# Autodesk Inventor assembly: arm
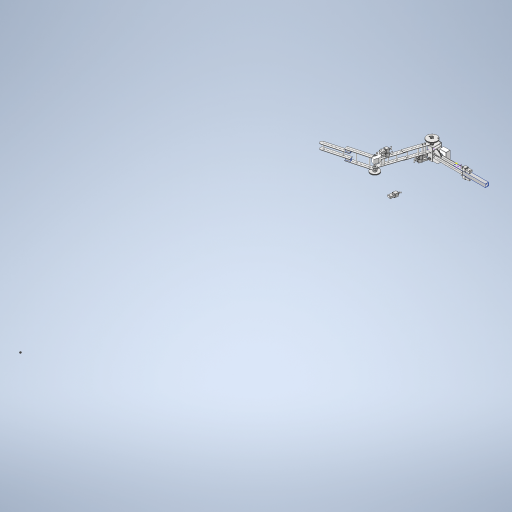
[picture p0: Inventor's stored thumbnail of the model, 512x512]
Saved by Autodesk Inventor 2024 (Build 280153000, 153)
## iProperties
Created: 2025-08-05
Part Number: arm
Document SubType Name: Assembly
Designer: HosodaLab2
Author: HosodaLab2
## iProperties of the stored document CSH-SUS-M6-130.ipt
Created: 2014-02-13
Part Number: CSH-SUS-M6-130
Material: 一般
Document SubType Name: Modeling
Designer: HosodaLab2
Density: 1 g/cm^3
Appearance: 既定
Sending System: SolidWorks 2007
Last Author: guan-li
Last Saved: 2014-03-10
Author: HosodaLab2
## Documents named in this file (68)
- C:\Users\HosodaLab2\OneDrive - Kyoto University\ドキュメント\Inventor\arm2\arm.iam
- C:\Users\HosodaLab2\OneDrive - Kyoto University\ドキュメント\Inventor\arm2\arm_jig.ipt
- C:\Users\HosodaLab2\OneDrive - Kyoto University\ドキュメント\Inventor\arm2\elbow_stopper.ipt
- C:\Users\HosodaLab2\OneDrive - Kyoto University\ドキュメント\Inventor\arm2\base.ipt
- C:\Users\HosodaLab2\OneDrive - Kyoto University\ドキュメント\Inventor\arm2\elbow_lower_plate.ipt
- C:\Users\HosodaLab2\OneDrive - Kyoto University\ドキュメント\Inventor\arm2\elbow_upper_plate.ipt
- C:\Users\HosodaLab2\OneDrive - Kyoto University\ドキュメント\Inventor\arm2\shoulder_stopper.ipt
- C:\Users\HosodaLab2\OneDrive - Kyoto University\ドキュメント\Inventor\arm2\CUI_AMT102-1024-I8000-S.iam
- C:\Users\HosodaLab2\OneDrive - Kyoto University\ドキュメント\Inventor\arm2\STHRANG8-MB.iam
- C:\Users\HosodaLab2\OneDrive - Kyoto University\ドキュメント\Inventor\arm2\F686ZZ.ipt
- C:\Users\HosodaLab2\OneDrive - Kyoto University\ドキュメント\Inventor\arm2\shoulder1_shaft.ipt
- C:\Users\HosodaLab2\OneDrive - Kyoto University\ドキュメント\Inventor\arm2\elbow_shaft.ipt
- C:\Users\HosodaLab2\OneDrive - Kyoto University\ドキュメント\Inventor\arm2\pully_elbow.ipt
- C:\Users\HosodaLab2\OneDrive - Kyoto University\ドキュメント\Inventor\arm2\pully_shoulder1.ipt
- C:\Users\HosodaLab2\OneDrive - Kyoto University\ドキュメント\Inventor\arm2\shoulder1_upper_plate.ipt
- C:\Users\HosodaLab2\OneDrive - Kyoto University\ドキュメント\Inventor\arm2\shoulder1_shaftholder_spacer_bottom.ipt
- C:\Users\HosodaLab2\OneDrive - Kyoto University\ドキュメント\Inventor\arm2\shoulder1_shaftholder_spacer_upper.ipt
- C:\Users\HosodaLab2\OneDrive - Kyoto University\ドキュメント\Inventor\arm2\shoulder1_upper_enocder_spacer.ipt
- C:\Users\HosodaLab2\OneDrive - Kyoto University\ドキュメント\Inventor\arm2\shoulder1_under_lower_plate_spacer.ipt
- C:\Users\HosodaLab2\OneDrive - Kyoto University\ドキュメント\Inventor\arm2\shoulder1_lower_cover.ipt
- C:\Users\HosodaLab2\OneDrive - Kyoto University\ドキュメント\Inventor\arm2\shoulder1_upper_cover.ipt
- C:\Users\HosodaLab2\OneDrive - Kyoto University\ドキュメント\Inventor\arm2\STHRANG10-MB_ss.ipt
- C:\Users\HosodaLab2\OneDrive - Kyoto University\ドキュメント\Inventor\arm2\shoulder1_lower_plate.ipt
- C:\Users\HosodaLab2\OneDrive - Kyoto University\ドキュメント\Inventor\arm2\F688ZZ.iam
- C:\Users\HosodaLab2\OneDrive - Kyoto University\ドキュメント\Inventor\arm2\SCST6-8.iam
- C:\Users\HosodaLab2\OneDrive - Kyoto University\ドキュメント\Inventor\arm2\shoulder2_upper_plate_spacer.ipt
- C:\Users\HosodaLab2\OneDrive - Kyoto University\ドキュメント\Inventor\arm2\shoulder1_encorder_spacer.ipt
- C:\Users\HosodaLab2\OneDrive - Kyoto University\ドキュメント\Inventor\arm2\shoulder2_pully_spacer.ipt
- C:\Users\HosodaLab2\OneDrive - Kyoto University\ドキュメント\Inventor\arm2\pully_shoulder2.ipt
- pully_shoulder_2_80.ipt
- C:\Users\HosodaLab2\OneDrive - Kyoto University\ドキュメント\Inventor\arm2\shoulder2_upperplate_left_spacer.ipt
- C:\Users\HosodaLab2\OneDrive - Kyoto University\ドキュメント\Inventor\arm2\shoulder2_upperplate_right_spacer.ipt
- C:\Users\HosodaLab2\OneDrive - Kyoto University\ドキュメント\Inventor\arm2\shoulder2_lower_left_plate.ipt
- C:\Users\HosodaLab2\OneDrive - Kyoto University\ドキュメント\Inventor\arm2\shoulder2_lower_right_plate.ipt
- C:\Users\HosodaLab2\OneDrive - Kyoto University\ドキュメント\Inventor\arm2\elbow_encorder_spacer.ipt
- C:\Users\HosodaLab2\OneDrive - Kyoto University\ドキュメント\Inventor\arm2\elbow_upperplate_left_spacer.ipt
- C:\Users\HosodaLab2\OneDrive - Kyoto University\ドキュメント\Inventor\arm2\elbow_upperplate_right_spacer.ipt
- C:\Users\HosodaLab2\OneDrive - Kyoto University\ドキュメント\Inventor\arm2\elbow_pully_spacer.ipt
- C:\Users\HosodaLab2\OneDrive - Kyoto University\ドキュメント\Inventor\arm2\shoulder2_lower_plate_spacer.ipt
- C:\Users\HosodaLab2\OneDrive - Kyoto University\ドキュメント\Inventor\arm2\elbow_lower_plate_spacer.ipt
- C:\Users\HosodaLab2\OneDrive - Kyoto University\ドキュメント\Inventor\arm2\elbow_upper_plate_spacer.ipt
- C:\Users\HosodaLab2\OneDrive - Kyoto University\ドキュメント\Inventor\arm2\shoulder1_NewPart2.ipt
- **C:\Users\HosodaLab2\OneDrive - Kyoto University\ドキュメント\Inventor\arm2\arm.iam*LocalDocs*xAaaaalcaAaaaaaaaAaaaqn4oUb*CSH-SUS-M6-130.ipt
- C:\Users\HosodaLab2\OneDrive - Kyoto University\ドキュメント\Inventor\arm2\shoulder2_elbow_strain_sensor_near.iam
- C:\Users\HosodaLab2\OneDrive - Kyoto University\ドキュメント\Inventor\arm2\shoulder2_elbow_strain_sensor_away.iam
- C:\Users\HosodaLab2\OneDrive - Kyoto University\ドキュメント\Inventor\arm2\shoulder2_shaft.ipt
- C:\Users\HosodaLab2\OneDrive - Kyoto University\ドキュメント\Inventor\arm2\shoulder2_lower_plate_bolt_spcaer.ipt
- C:\Users\HosodaLab2\OneDrive - Kyoto University\ドキュメント\Inventor\arm2\shoulder2_uppper_plate_bolt_spcaer.ipt
- C:\Users\HosodaLab2\OneDrive - Kyoto University\ドキュメント\Inventor\arm2\strain_sensor_spacer.ipt
- C:\Users\HosodaLab2\OneDrive - Kyoto University\ドキュメント\Inventor\arm2\shoulder1_strain_sensor.iam
- C:\Users\HosodaLab2\OneDrive - Kyoto University\ドキュメント\Inventor\arm2\shoulder1_strain_sensor_spacer.ipt
- C:\Users\HosodaLab2\OneDrive - Kyoto University\ドキュメント\Inventor\arm2\shoulder2_shaftholder_spacer_upper.ipt
- C:\Users\HosodaLab2\OneDrive - Kyoto University\ドキュメント\Inventor\arm2\3dprint\pully_elbow_40.ipt
- C:\Users\HosodaLab2\OneDrive - Kyoto University\ドキュメント\Inventor\arm2\3dprint\pully_elbow_50.ipt
- C:\Users\HosodaLab2\OneDrive - Kyoto University\ドキュメント\Inventor\arm2\SCST8-8.iam
- C:\Users\HosodaLab2\OneDrive - Kyoto University\ドキュメント\Inventor\arm2\shoulder2_upper_plate_left.ipt
- C:\Users\HosodaLab2\OneDrive - Kyoto University\ドキュメント\Inventor\arm2\shoulder2_upper_plate_rigth.ipt
- shoulder2_upper_plate_rigtht.ipt
- C:\Users\HosodaLab2\OneDrive - Kyoto University\ドキュメント\Inventor\arm2\shoulder2_encorder_spacer.ipt
- C:\Users\HosodaLab2\OneDrive - Kyoto University\ドキュメント\Inventor\arm2\shoulder2_shaftholder_spacer.ipt
- C:\Users\HosodaLab2\OneDrive - Kyoto University\ドキュメント\Inventor\arm2\shoulder1_verticval_cover.ipt
- C:\Users\HosodaLab2\OneDrive - Kyoto University\ドキュメント\Inventor\arm2\pully_shoulder2_70.ipt
- C:\Users\HosodaLab2\OneDrive - Kyoto University\ドキュメント\Inventor\arm2\pully_shoulder2_90ipt.ipt
- C:\Users\HosodaLab2\OneDrive - Kyoto University\ドキュメント\Inventor\arm2\pully_shoulder2_100.ipt
- C:\Users\HosodaLab2\OneDrive - Kyoto University\ドキュメント\Inventor\Content Center Files\R2024\ja-JP\ISO 4762(2)\ISO 4762 - M3 x 16ISO.ipt
- C:\Users\HosodaLab2\OneDrive - Kyoto University\ドキュメント\Inventor\arm2\new_shoulder2_elbow_strain_sensor_away.iam
- **C:\Users\HosodaLab2\OneDrive - Kyoto University\ドキュメント\Inventor\arm\arm.iam*LocalDocs*xAaaaalcaAaaaaaaaAaaaqn4oUb*CSH-SUS-M6-130.ipt
- C:\Users\HosodaLab2\OneDrive - Kyoto University\ドキュメント\Inventor\arm2\CSH-SUS-M6-130.SLDPRT
## Components (102 placed, 60 different names)
1. arm_jig:1 — 回転:140, 回転:141, 回転:142, 回転:143
2. base:1 — 回転:34, 回転:74, 回転:217, 回転:218, 円柱状:21, 円柱状:22, メイト:10, 円柱状:23, 円柱状:24, メイト:11, 回転:225, 回転:226, 回転:227, 回転:228
3. elbow_lower_plate:1 — 回転:142, 回転:143, リジッド:2, 回転:167
4. elbow_stopper:1 — 回転:168, 回転:169
5. shoulder1_encorder_spacer:1 — 回転:62, 回転:63
6. shoulder_stopper:1 — 回転:58, 回転:59
7. shoulder1_plate:1 — 回転:34, 角度:3, 回転:58, 回転:59, 回転:62, 回転:63, 回転:89, 角度:5, 回転:217
8. elbow_upper_plate:2 — 回転:140, 回転:141, 回転:144, 回転:153, 回転:215, 回転:216
9. shoulder2_lower_left_plate:1 — 回転:132, 回転:133, 角度:9, 回転:152, 回転:182, 回転:183, 回転:184, 回転:185, 回転:219
10. shoulder2_upper_plate_left:1 — 回転:173, 回転:175, メイト:3, 回転:184, 回転:185, 回転:220, 回転:263
11. shoulder2_lower_right_plate:1 — 回転:106, 回転:151, 回転:168, 回転:169, メイト:5, 回転:186, 回転:187, 回転:190
12. shoulder2_upper_plate_rigtht:1 — 回転:186, 回転:187, 回転:200, 回転:201, 回転:202, 回転:203, 回転:245, 回転:262, 回転:266, 回転:267, 角度:10
13. arm_jig:2
14. elbow_lower_plate:3 — 回転:155, 回転:156
15. elbow_upper_plate:3 — 回転:154, 回転:161, 回転:162, 回転:163, 回転:166, リジッド:1
16. CUI_AMT102-1024-I8000-S:3 [sub-assembly] — 角度:3, 回転:87, 回転:92
17. F686ZZ:1
18. pully_elbow:1 — 回転:164, 回転:165
19. pully_shoulder1:3 — 回転:157, 回転:158
20. shoulder1_shaftholder_spacer_bottom:1 — 回転:79, 回転:121
21. shoulder1_shaftholder_spacer_upper:1 — 回転:83
22. shoulder1_upper_enocder_spacer:1 — 回転:87, 回転:95
23. shoulder1_under_lower_plate_spacer:1 — 回転:93, 回転:109
24. shoulder1_upper_cover:1 — 角度:5, 回転:95, 回転:231, 回転:235, 回転:236, 回転:274, 回転:275
25. shoulder1_verticval_cover:1 — 回転:235, 回転:236, 回転:237, 回転:238, 回転:259, 回転:282, メイト:16, メイト:18, メイト:20, 回転:283
26. STHRANG10-MB_ss:1 — 回転:79, 回転:83, 回転:157, 回転:158, メイト:9
27. STHRANG8-MB:2 [sub-assembly] — 円柱状:8, 回転:159, 回転:253, 回転:281, メイト:15
28. shoulder1_lower_plate:1 — 回転:74, 回転:88, 角度:7, 回転:218
29. F688ZZ:1 [sub-assembly] — 回転:88, 回転:93, 回転:121, 回転:211
30. shoulder2_upper_plate_spacer:1 — 回転:173, 回転:200
31. F688ZZ:3 [sub-assembly] — 回転:106, 回転:137
32. F688ZZ:4 [sub-assembly] — 回転:134, 回転:212
33. shoulder1_lower_cover:2 — 角度:7, 回転:109, 回転:237, 回転:238, 回転:242, 回転:243, 回転:244
34. pully_shoulder_2_80:1 — 円柱状:8, 回転:159
35. CUI_AMT102-1024-I8000-S:4 [sub-assembly] — 回転:134, 角度:9, 回転:136
36. elbow_encorder_spacer:1 — 回転:132, 回転:133
37. elbow_upperplate_right_spacer:1 — 回転:137, 回転:144
38. elbow_upperplate_left_spacer:2 — 回転:136, 回転:162
39. elbow_pully_spacer:1 — 回転:146, 回転:147, 回転:161, 回転:163
40. STHRANG8-MB:4 [sub-assembly] — 回転:146, 回転:147, 回転:164, 回転:165, メイト:7
41. STHRANG8-MB:5 [sub-assembly] — 回転:215, 回転:216
42. shoulder2_upper_plate_spacer:2 — 回転:175
43. shoulder2_lower_plate_spacer:1 — 回転:151
44. shoulder2_lower_plate_spacer:2 — 回転:152
45. elbow_lower_plate_spacer:1 — 回転:155, リジッド:2
46. elbow_upper_plate_spacer:1 — 回転:153, 回転:166
47. elbow_upper_plate_spacer:2 — 回転:154, リジッド:1
48. elbow_lower_plate_spacer:2 — 回転:156, 回転:167
49. shoulder1_NewPart2:1
50. shoulder2_elbow_strain_sensor_near:1 [sub-assembly] — メイト:3, メイト:4, 円柱状:17, 円柱状:18, 回転:222
51. CSH-SUS-M6-130:1 — 回転:202, 円柱状:18, 円柱状:20
52. CSH-SUS-M6-130:2 — 回転:201, 円柱状:17, 円柱状:19
53. CSH-SUS-M6-130:3 — 回転:183, 円柱状:14, 円柱状:16
54. CSH-SUS-M6-130:4 — 回転:182, 円柱状:13, 円柱状:15
55. shoulder2_elbow_strain_sensor_away:1 [sub-assembly] — メイト:4, 円柱状:19, 円柱状:20, 回転:221
56. shoulder2_elbow_strain_sensor_away:2 [sub-assembly] — 円柱状:15, 円柱状:16, メイト:6
57. shoulder2_elbow_strain_sensor_near:2 [sub-assembly] — 円柱状:13, 円柱状:14, メイト:5, メイト:6, 回転:223, 回転:224
58. shoulder2_uppper_plate_bolt_spcaer:1 — 回転:203
59. shoulder2_lower_plate_bolt_spcaer:1 — 回転:190
60. shoulder1_shaft:1 — 回転:211, メイト:9, 円柱状:25, 回転:241
61. elbow_shaft:1 — 回転:212, メイト:7
62. shoulder2_shaft:1 — 回転:282, 円柱状:26, 円柱状:27, メイト:15
63. shoulder2_lower_plate_bolt_spcaer:2 — 回転:219
64. shoulder2_uppper_plate_bolt_spcaer:2 — 回転:220
65. strain_sensor_spacer:1 — 回転:221
66. strain_sensor_spacer:2 — 回転:222
67. strain_sensor_spacer:3 — 回転:223
68. strain_sensor_spacer:4 — 回転:224
69. shoulder1_strain_sensor:1 [sub-assembly] — 円柱状:21, 円柱状:22, メイト:10
70. shoulder1_strain_sensor:2 [sub-assembly] — 円柱状:23, 円柱状:24, メイト:11
71. shoulder1_strain_sensor_spacer:1 — 回転:225
72. shoulder1_strain_sensor_spacer:2 — 回転:228
73. shoulder1_strain_sensor_spacer:3 — 回転:226
74. shoulder1_strain_sensor_spacer:4 — 回転:227
75. F688ZZ:2 [sub-assembly] — 回転:89, 回転:92
76. STHRANG8-MB:6 [sub-assembly] — 円柱状:25, 回転:231
77. shoulder2_shaftholder_spacer_upper:1
78. STHRANG8-MB:9 [sub-assembly] — 回転:241, 回転:242
79. SCST6-8:1 [sub-assembly] — 回転:243, 回転:244
80. pully_elbow_40:1
81. pully_elbow_50:1
82. SCST8-8:1 [sub-assembly] — 回転:259, メイト:12, メイト:13, メイト:17, メイト:19, メイト:21, 回転:283
83. CUI_AMT102-1024-I8000-S:5 [sub-assembly] — 回転:245, 回転:246, 回転:268, 角度:10
84. F688ZZ:7 [sub-assembly] — 回転:262, 回転:265, 回転:268
85. shoulder2_pully_spacer:2 — 回転:246, 回転:253
86. shoulder2_upperplate_left_spacer:2 — 回転:279, 円柱状:27
87. shoulder2_upperplate_right_spacer:2 — 回転:265, メイト:12, 円柱状:26, メイト:13
88. SCST8-8:2 [sub-assembly] — 回転:276, 回転:278
89. F688ZZ:9 [sub-assembly] — 回転:263, 回転:264, 回転:271, 回転:273, 回転:279
90. STHRANG8-MB:10 [sub-assembly] — 回転:264
91. shoulder2_encorder_spacer:1 — 回転:266, 回転:267
92. shoulder2_shaftholder_spacer:1 — 回転:271
93. SCST8-8:3 [sub-assembly] — 回転:273
94. shoulder1_verticval_cover:2 — 回転:274, 回転:275, 回転:276, 回転:278
95. SCST8-8:4 [sub-assembly] — 回転:281
96. pully_shoulder_2_80:6
97. pully_shoulder_2_80:5
98. pully_shoulder_2_80:7
99. ISO 4762 M3 x 16:1 — メイト:16, メイト:17
100. ISO 4762 M3 x 16:2 — メイト:18, メイト:19
101. ISO 4762 M3 x 16:3 — メイト:20, メイト:21
102. new_shoulder2_elbow_strain_sensor_away:1 [sub-assembly]
## Relationships (150: RevoluteJoint 110, Mate 17, CylindricalJoint 16, Angle 5, WeldJoint 2)
- [RevoluteJoint]: arm_jig:2 ↔ elbow_upper_plate:3
- [RevoluteJoint]: arm_jig:2 ↔ elbow_upper_plate:3
- [RevoluteJoint]: arm_jig:2 ↔ elbow_lower_plate:3
- [RevoluteJoint]: arm_jig:2 ↔ elbow_lower_plate:3
- 回転:34 [RevoluteJoint]: base:1 ↔ shoulder1_plate:1
- 角度:3 [Angle] (180 deg): shoulder1_plate:1 ↔ CUI_AMT102-1024-I8000-S:3
- 回転:58 [RevoluteJoint]: shoulder_stopper:1 ↔ shoulder1_plate:1
- 回転:59 [RevoluteJoint]: shoulder_stopper:1 ↔ shoulder1_plate:1
- 回転:62 [RevoluteJoint]: shoulder1_encorder_spacer:1 ↔ shoulder1_plate:1
- 回転:63 [RevoluteJoint]: shoulder1_encorder_spacer:1 ↔ shoulder1_plate:1
- 回転:74 [RevoluteJoint]: base:1 ↔ shoulder1_lower_plate:1
- 回転:79 [RevoluteJoint]: shoulder1_shaftholder_spacer_bottom:1 ↔ STHRANG10-MB_ss:1
- 回転:83 [RevoluteJoint]: shoulder1_shaftholder_spacer_upper:1 ↔ STHRANG10-MB_ss:1
- 回転:87 [RevoluteJoint]: CUI_AMT102-1024-I8000-S:3 ↔ shoulder1_upper_enocder_spacer:1
- 回転:88 [RevoluteJoint]: shoulder1_lower_plate:1 ↔ F688ZZ:1
- 回転:89 [RevoluteJoint]: shoulder1_plate:1 ↔ F688ZZ:2
- 角度:5 [Angle] (0 deg): shoulder1_plate:1 ↔ shoulder1_upper_cover:1
- 回転:92 [RevoluteJoint]: CUI_AMT102-1024-I8000-S:3 ↔ F688ZZ:2
- 回転:93 [RevoluteJoint]: shoulder1_under_lower_plate_spacer:1 ↔ F688ZZ:1
- 回転:95 [RevoluteJoint]: shoulder1_upper_enocder_spacer:1 ↔ shoulder1_upper_cover:1
- 回転:106 [RevoluteJoint]: shoulder2_lower_right_plate:1 ↔ F688ZZ:3
- 角度:7 [Angle] (180 deg): shoulder1_lower_plate:1 ↔ shoulder1_lower_cover:2
- 回転:109 [RevoluteJoint]: shoulder1_under_lower_plate_spacer:1 ↔ shoulder1_lower_cover:2
- 回転:121 [RevoluteJoint]: shoulder1_shaftholder_spacer_bottom:1 ↔ F688ZZ:1
- 回転:132 [RevoluteJoint]: shoulder2_lower_left_plate:1 ↔ elbow_encorder_spacer:1
- 回転:133 [RevoluteJoint]: shoulder2_lower_left_plate:1 ↔ elbow_encorder_spacer:1
- 回転:134 [RevoluteJoint]: F688ZZ:4 ↔ CUI_AMT102-1024-I8000-S:4
- 角度:9 [Angle] (0 deg): shoulder2_lower_left_plate:1 ↔ CUI_AMT102-1024-I8000-S:4
- 回転:136 [RevoluteJoint]: CUI_AMT102-1024-I8000-S:4 ↔ elbow_upperplate_left_spacer:2
- 回転:137 [RevoluteJoint]: F688ZZ:3 ↔ elbow_upperplate_right_spacer:1
- 回転:140 [RevoluteJoint]: arm_jig:1 ↔ elbow_upper_plate:2
- 回転:141 [RevoluteJoint]: arm_jig:1 ↔ elbow_upper_plate:2
- 回転:142 [RevoluteJoint]: arm_jig:1 ↔ elbow_lower_plate:1
- 回転:143 [RevoluteJoint]: arm_jig:1 ↔ elbow_lower_plate:1
- 回転:144 [RevoluteJoint]: elbow_upper_plate:2 ↔ elbow_upperplate_right_spacer:1
- 回転:146 [RevoluteJoint]: elbow_pully_spacer:1 ↔ STHRANG8-MB:4
- 回転:147 [RevoluteJoint]: elbow_pully_spacer:1 ↔ STHRANG8-MB:4
- 回転:151 [RevoluteJoint]: shoulder2_lower_right_plate:1 ↔ shoulder2_lower_plate_spacer:1
- 回転:152 [RevoluteJoint]: shoulder2_lower_left_plate:1 ↔ shoulder2_lower_plate_spacer:2
- 回転:153 [RevoluteJoint]: elbow_upper_plate:2 ↔ elbow_upper_plate_spacer:1
- 回転:154 [RevoluteJoint]: elbow_upper_plate:3 ↔ elbow_upper_plate_spacer:2
- 回転:155 [RevoluteJoint]: elbow_lower_plate:3 ↔ elbow_lower_plate_spacer:1
- 回転:156 [RevoluteJoint]: elbow_lower_plate:3 ↔ elbow_lower_plate_spacer:2
- 回転:157 [RevoluteJoint]: pully_shoulder1:3 ↔ STHRANG10-MB_ss:1
- 回転:158 [RevoluteJoint]: pully_shoulder1:3 ↔ STHRANG10-MB_ss:1
- 円柱状:8 [CylindricalJoint]: STHRANG8-MB:2 ↔ pully_shoulder_2_80:1
- 回転:159 [RevoluteJoint]: STHRANG8-MB:2 ↔ pully_shoulder_2_80:1
- 回転:161 [RevoluteJoint]: elbow_upper_plate:3 ↔ elbow_pully_spacer:1
- 回転:162 [RevoluteJoint]: elbow_upper_plate:3 ↔ elbow_upperplate_left_spacer:2
- 回転:163 [RevoluteJoint]: elbow_upper_plate:3 ↔ elbow_pully_spacer:1
- 回転:164 [RevoluteJoint]: pully_elbow:1 ↔ STHRANG8-MB:4
- 回転:165 [RevoluteJoint]: pully_elbow:1 ↔ STHRANG8-MB:4
- 回転:166 [RevoluteJoint]: elbow_upper_plate:3 ↔ elbow_upper_plate_spacer:1
- リジッド:1 [WeldJoint]: elbow_upper_plate:3 ↔ elbow_upper_plate_spacer:2
- リジッド:2 [WeldJoint]: elbow_lower_plate:1 ↔ elbow_lower_plate_spacer:1
- 回転:167 [RevoluteJoint]: elbow_lower_plate:1 ↔ elbow_lower_plate_spacer:2
- 回転:168 [RevoluteJoint]: elbow_stopper:1 ↔ shoulder2_lower_right_plate:1
- 回転:169 [RevoluteJoint]: elbow_stopper:1 ↔ shoulder2_lower_right_plate:1
- 回転:173 [RevoluteJoint]: shoulder2_upper_plate_left:1 ↔ shoulder2_upper_plate_spacer:1
- 回転:175 [RevoluteJoint]: shoulder2_upper_plate_left:1 ↔ shoulder2_upper_plate_spacer:2
- 回転:182 [RevoluteJoint]: shoulder2_lower_left_plate:1 ↔ CSH-SUS-M6-130:4
- 回転:183 [RevoluteJoint]: shoulder2_lower_left_plate:1 ↔ CSH-SUS-M6-130:3
- メイト:3 [Mate] (3 mm): shoulder2_upper_plate_left:1 ↔ shoulder2_elbow_strain_sensor_near:1
- メイト:4 [Mate]: shoulder2_elbow_strain_sensor_near:1 ↔ shoulder2_elbow_strain_sensor_away:1
- 円柱状:13 [CylindricalJoint]: CSH-SUS-M6-130:4 ↔ shoulder2_elbow_strain_sensor_near:2
- 円柱状:14 [CylindricalJoint]: CSH-SUS-M6-130:3 ↔ shoulder2_elbow_strain_sensor_near:2
- メイト:5 [Mate] (3 mm): shoulder2_lower_right_plate:1 ↔ shoulder2_elbow_strain_sensor_near:2
- 円柱状:15 [CylindricalJoint]: CSH-SUS-M6-130:4 ↔ shoulder2_elbow_strain_sensor_away:2
- 円柱状:16 [CylindricalJoint]: CSH-SUS-M6-130:3 ↔ shoulder2_elbow_strain_sensor_away:2
- メイト:6 [Mate]: shoulder2_elbow_strain_sensor_away:2 ↔ shoulder2_elbow_strain_sensor_near:2
- 回転:184 [RevoluteJoint]: shoulder2_lower_left_plate:1 ↔ shoulder2_upper_plate_left:1
- 回転:185 [RevoluteJoint]: shoulder2_lower_left_plate:1 ↔ shoulder2_upper_plate_left:1
- 回転:186 [RevoluteJoint]: shoulder2_lower_right_plate:1 ↔ shoulder2_upper_plate_rigtht:1
- 回転:187 [RevoluteJoint]: shoulder2_lower_right_plate:1 ↔ shoulder2_upper_plate_rigtht:1
- 回転:190 [RevoluteJoint]: shoulder2_lower_right_plate:1 ↔ shoulder2_lower_plate_bolt_spcaer:1
- 回転:200 [RevoluteJoint]: shoulder2_upper_plate_rigtht:1 ↔ shoulder2_upper_plate_spacer:1
- 回転:201 [RevoluteJoint]: shoulder2_upper_plate_rigtht:1 ↔ CSH-SUS-M6-130:2
- 回転:202 [RevoluteJoint]: shoulder2_upper_plate_rigtht:1 ↔ CSH-SUS-M6-130:1
- 円柱状:17 [CylindricalJoint]: shoulder2_elbow_strain_sensor_near:1 ↔ CSH-SUS-M6-130:2
- 円柱状:18 [CylindricalJoint]: shoulder2_elbow_strain_sensor_near:1 ↔ CSH-SUS-M6-130:1
- 円柱状:19 [CylindricalJoint]: CSH-SUS-M6-130:2 ↔ shoulder2_elbow_strain_sensor_away:1
- 円柱状:20 [CylindricalJoint]: CSH-SUS-M6-130:1 ↔ shoulder2_elbow_strain_sensor_away:1
- 回転:203 [RevoluteJoint]: shoulder2_upper_plate_rigtht:1 ↔ shoulder2_uppper_plate_bolt_spcaer:1
- 回転:211 [RevoluteJoint]: F688ZZ:1 ↔ shoulder1_shaft:1
- 回転:212 [RevoluteJoint]: F688ZZ:4 ↔ elbow_shaft:1
- メイト:7 [Mate]: STHRANG8-MB:4 ↔ elbow_shaft:1
- 回転:215 [RevoluteJoint]: elbow_upper_plate:2 ↔ STHRANG8-MB:5
- 回転:216 [RevoluteJoint]: elbow_upper_plate:2 ↔ STHRANG8-MB:5
- メイト:9 [Mate]: STHRANG10-MB_ss:1 ↔ shoulder1_shaft:1
- 回転:217 [RevoluteJoint]: base:1 ↔ shoulder1_plate:1
- 回転:218 [RevoluteJoint]: base:1 ↔ shoulder1_lower_plate:1
- 回転:219 [RevoluteJoint]: shoulder2_lower_left_plate:1 ↔ shoulder2_lower_plate_bolt_spcaer:2
- 回転:220 [RevoluteJoint]: shoulder2_upper_plate_left:1 ↔ shoulder2_uppper_plate_bolt_spcaer:2
- 回転:221 [RevoluteJoint]: shoulder2_elbow_strain_sensor_away:1 ↔ strain_sensor_spacer:1
- 回転:222 [RevoluteJoint]: shoulder2_elbow_strain_sensor_near:1 ↔ strain_sensor_spacer:2
- 回転:223 [RevoluteJoint]: shoulder2_elbow_strain_sensor_near:2 ↔ strain_sensor_spacer:3
- 回転:224 [RevoluteJoint]: shoulder2_elbow_strain_sensor_near:2 ↔ strain_sensor_spacer:4
- 円柱状:21 [CylindricalJoint]: base:1 ↔ shoulder1_strain_sensor:1
- 円柱状:22 [CylindricalJoint]: base:1 ↔ shoulder1_strain_sensor:1
- メイト:10 [Mate]: base:1 ↔ shoulder1_strain_sensor:1
- 円柱状:23 [CylindricalJoint]: base:1 ↔ shoulder1_strain_sensor:2
- 円柱状:24 [CylindricalJoint]: base:1 ↔ shoulder1_strain_sensor:2
- メイト:11 [Mate]: base:1 ↔ shoulder1_strain_sensor:2
- 回転:225 [RevoluteJoint]: base:1 ↔ shoulder1_strain_sensor_spacer:1
- 回転:226 [RevoluteJoint]: base:1 ↔ shoulder1_strain_sensor_spacer:3
- 回転:227 [RevoluteJoint]: base:1 ↔ shoulder1_strain_sensor_spacer:4
- 回転:228 [RevoluteJoint]: base:1 ↔ shoulder1_strain_sensor_spacer:2
- 円柱状:25 [CylindricalJoint]: shoulder1_shaft:1 ↔ STHRANG8-MB:6
- 回転:231 [RevoluteJoint]: shoulder1_upper_cover:1 ↔ STHRANG8-MB:6
- 回転:235 [RevoluteJoint]: shoulder1_upper_cover:1 ↔ shoulder1_verticval_cover:1
- 回転:236 [RevoluteJoint]: shoulder1_upper_cover:1 ↔ shoulder1_verticval_cover:1
- 回転:237 [RevoluteJoint]: shoulder1_verticval_cover:1 ↔ shoulder1_lower_cover:2
- 回転:238 [RevoluteJoint]: shoulder1_verticval_cover:1 ↔ shoulder1_lower_cover:2
- 回転:241 [RevoluteJoint]: shoulder1_shaft:1 ↔ STHRANG8-MB:9
- 回転:242 [RevoluteJoint]: shoulder1_lower_cover:2 ↔ STHRANG8-MB:9
- 回転:243 [RevoluteJoint]: shoulder1_lower_cover:2 ↔ SCST6-8:1
- 回転:244 [RevoluteJoint]: shoulder1_lower_cover:2 ↔ SCST6-8:1
- 回転:245 [RevoluteJoint]: shoulder2_upper_plate_rigtht:1 ↔ CUI_AMT102-1024-I8000-S:5
- 回転:246 [RevoluteJoint]: CUI_AMT102-1024-I8000-S:5 ↔ shoulder2_pully_spacer:2
- 回転:253 [RevoluteJoint]: STHRANG8-MB:2 ↔ shoulder2_pully_spacer:2
- 回転:259 [RevoluteJoint]: shoulder1_verticval_cover:1 ↔ SCST8-8:1
- 回転:262 [RevoluteJoint]: shoulder2_upper_plate_rigtht:1 ↔ F688ZZ:7
- 回転:263 [RevoluteJoint]: shoulder2_upper_plate_left:1 ↔ F688ZZ:9
- 回転:264 [RevoluteJoint]: F688ZZ:9 ↔ STHRANG8-MB:10
- 回転:265 [RevoluteJoint]: F688ZZ:7 ↔ shoulder2_upperplate_right_spacer:2
- 回転:266 [RevoluteJoint]: shoulder2_upper_plate_rigtht:1 ↔ shoulder2_encorder_spacer:1
- 回転:267 [RevoluteJoint]: shoulder2_upper_plate_rigtht:1 ↔ shoulder2_encorder_spacer:1
- 回転:268 [RevoluteJoint]: CUI_AMT102-1024-I8000-S:5 ↔ F688ZZ:7
- 角度:10 [Angle] (0 deg): shoulder2_upper_plate_rigtht:1 ↔ CUI_AMT102-1024-I8000-S:5
- 回転:271 [RevoluteJoint]: F688ZZ:9 ↔ shoulder2_shaftholder_spacer:1
- 回転:273 [RevoluteJoint]: F688ZZ:9 ↔ SCST8-8:3
- 回転:274 [RevoluteJoint]: shoulder1_upper_cover:1 ↔ shoulder1_verticval_cover:2
- 回転:275 [RevoluteJoint]: shoulder1_upper_cover:1 ↔ shoulder1_verticval_cover:2
- 回転:276 [RevoluteJoint]: SCST8-8:2 ↔ shoulder1_verticval_cover:2
- 回転:278 [RevoluteJoint]: SCST8-8:2 ↔ shoulder1_verticval_cover:2
- 回転:279 [RevoluteJoint]: shoulder2_upperplate_left_spacer:2 ↔ F688ZZ:9
- メイト:12 [Mate] (3 mm): SCST8-8:1 ↔ shoulder2_upperplate_right_spacer:2
- 回転:281 [RevoluteJoint]: STHRANG8-MB:2 ↔ SCST8-8:4
- 回転:282 [RevoluteJoint]: shoulder1_verticval_cover:1 ↔ shoulder2_shaft:1
- 円柱状:26 [CylindricalJoint]: shoulder2_shaft:1 ↔ shoulder2_upperplate_right_spacer:2
- メイト:13 [Mate] (3 mm): SCST8-8:1 ↔ shoulder2_upperplate_right_spacer:2
- 円柱状:27 [CylindricalJoint]: shoulder2_shaft:1 ↔ shoulder2_upperplate_left_spacer:2
- メイト:15 [Mate]: STHRANG8-MB:2 ↔ shoulder2_shaft:1
- メイト:16 [Mate]: shoulder1_verticval_cover:1 ↔ ISO 4762 M3 x 16:1
- メイト:17 [Mate]: SCST8-8:1 ↔ ISO 4762 M3 x 16:1
- メイト:18 [Mate]: shoulder1_verticval_cover:1 ↔ ISO 4762 M3 x 16:2
- メイト:19 [Mate]: SCST8-8:1 ↔ ISO 4762 M3 x 16:2
- メイト:20 [Mate]: shoulder1_verticval_cover:1 ↔ ISO 4762 M3 x 16:3
- メイト:21 [Mate]: SCST8-8:1 ↔ ISO 4762 M3 x 16:3
- 回転:283 [RevoluteJoint]: shoulder1_verticval_cover:1 ↔ SCST8-8:1
## Named parameters: d38_d30 = 0 mm, d39_d31 = 90 deg, d40_d32 = 0 mm, d41_d33 = 90 deg, d42_d34 = 0 mm, d43_d35 = 180 deg, d44_d36 = 0 mm, d45_d37 = -90 deg
